# Autodesk Inventor assembly: Aux Cooling Assembly
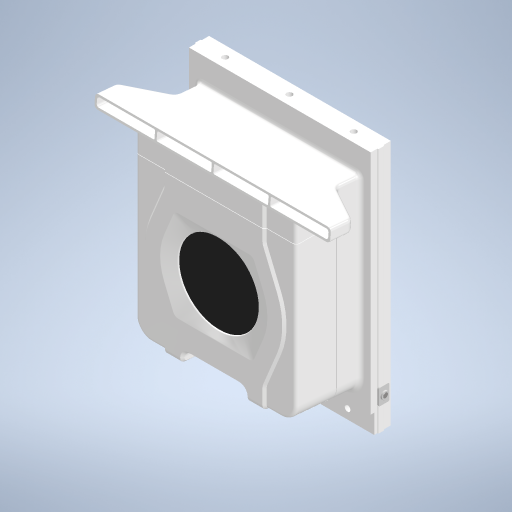
[picture p0: Inventor's stored thumbnail of the model, 512x512]
Saved by Autodesk Inventor 2024 (Build 280153000, 153)
## iProperties
Created: 2024-09-08
Part Number: Aux Cooling Assembly
Document SubType Name: Assembly
Designer: Ishaan
Author: Ishaan
## Documents named in this file (10)
- E:\Projects\Axiom--IDEX-3D-Printer\CAD\07 - Auxiliary Cooling\Aux Cooling Assembly.iam
- E:\Projects\Axiom--IDEX-3D-Printer\CAD\07 - Auxiliary Cooling\Aux Cooling Case.ipt
- E:\Projects\Axiom--IDEX-3D-Printer\CAD\00 - COTS Components\12032 Fan\SanAce_9BFB_120x32_BLW\SanAce_9BFB_120x32_BLW.ipt
- E:\Projects\Axiom--IDEX-3D-Printer\CAD\00 - COTS Components\HEPA Filter.ipt
- E:\Projects\Axiom--IDEX-3D-Printer\CAD\00 - COTS Components\Hardware\SHCSM5x20.ipt
- E:\Projects\Axiom--IDEX-3D-Printer\CAD\00 - COTS Components\Hardware\M5 LOCKNUT.ipt
- E:\Projects\Axiom--IDEX-3D-Printer\CAD\00 - COTS Components\Hardware\SHCSM5x16.ipt
- E:\Projects\Axiom--IDEX-3D-Printer\CAD\00 - COTS Components\Hardware\M5 T SLOT NUT.ipt
- E:\Projects\Axiom--IDEX-3D-Printer\CAD\00 - COTS Components\Hardware\SHCSM4x14.ipt
- E:\Projects\Axiom--IDEX-3D-Printer\CAD\00 - COTS Components\Hardware\M4 LOCKNUT.ipt
## Components (20 placed, 9 different names)
1. Aux Cooling Case:1 — Insert:1, Insert:2, Insert:3, Mate:1, Mate:2, Mate:3, Insert:4, Insert:5, Insert:6, Angle:1, Insert:7, Angle:2, Insert:8, Insert:9, Insert:10, Angle:3, Insert:11, Angle:4, Insert:12, Insert:13, Insert:14, Insert:18, Insert:19, Insert:20, Angle:5, Angle:6, Angle:7
2. SanAce_9BFB_120x32_BLW:1 — Insert:1, Insert:2, Insert:3, Insert:15, Insert:16, Insert:17
3. HEPA Filter:1 — Mate:1, Mate:2, Mate:3
4. SHCSM5x20:1 — Insert:4
5. SHCSM5x20:2 — Insert:5
6. M5 LOCKNUT:1 — Insert:7, Angle:2
7. M5 LOCKNUT:2 — Insert:6, Angle:1
8. SHCSM5x16:1 — Insert:8
9. SHCSM5x16:2 — Insert:9
10. M5 T SLOT NUT:1 — Insert:10, Angle:3
11. M5 T SLOT NUT:2 — Insert:11, Angle:4
12. SHCSM4x14:1 — Insert:12
13. SHCSM4x14:2 — Insert:13
14. SHCSM4x14:3 — Insert:14
15. M4 LOCKNUT:1 — Insert:15
16. M4 LOCKNUT:2 — Insert:17
17. M4 LOCKNUT:3 — Insert:16
18. M5 LOCKNUT:3 — Insert:20, Angle:5
19. M5 LOCKNUT:4 — Insert:19, Angle:6
20. M5 LOCKNUT:5 — Insert:18, Angle:7
## Relationships (30: Insert 20, Angle 7, Mate 3)
- Insert:1: Aux Cooling Case:1 ↔ SanAce_9BFB_120x32_BLW:1
- Insert:2: Aux Cooling Case:1 ↔ SanAce_9BFB_120x32_BLW:1
- Insert:3: Aux Cooling Case:1 ↔ SanAce_9BFB_120x32_BLW:1
- Mate:1 (0.5 mm): Aux Cooling Case:1 ↔ HEPA Filter:1
- Mate:2 (0.25 mm): Aux Cooling Case:1 ↔ HEPA Filter:1
- Mate:3 (0.5 mm): Aux Cooling Case:1 ↔ HEPA Filter:1
- Insert:4: Aux Cooling Case:1 ↔ SHCSM5x20:1
- Insert:5: Aux Cooling Case:1 ↔ SHCSM5x20:2
- Insert:6: Aux Cooling Case:1 ↔ M5 LOCKNUT:2
- Angle:1 (0 deg): Aux Cooling Case:1 ↔ M5 LOCKNUT:2
- Insert:7: Aux Cooling Case:1 ↔ M5 LOCKNUT:1
- Angle:2 (0 deg): Aux Cooling Case:1 ↔ M5 LOCKNUT:1
- Insert:8: Aux Cooling Case:1 ↔ SHCSM5x16:1
- Insert:9: Aux Cooling Case:1 ↔ SHCSM5x16:2
- Insert:10 (2 mm): Aux Cooling Case:1 ↔ M5 T SLOT NUT:1
- Angle:3 (0 deg): Aux Cooling Case:1 ↔ M5 T SLOT NUT:1
- Insert:11 (2 mm): Aux Cooling Case:1 ↔ M5 T SLOT NUT:2
- Angle:4 (0 deg): Aux Cooling Case:1 ↔ M5 T SLOT NUT:2
- Insert:12: Aux Cooling Case:1 ↔ SHCSM4x14:1
- Insert:13: Aux Cooling Case:1 ↔ SHCSM4x14:2
- Insert:14: Aux Cooling Case:1 ↔ SHCSM4x14:3
- Insert:15: SanAce_9BFB_120x32_BLW:1 ↔ M4 LOCKNUT:1
- Insert:16: SanAce_9BFB_120x32_BLW:1 ↔ M4 LOCKNUT:3
- Insert:17: SanAce_9BFB_120x32_BLW:1 ↔ M4 LOCKNUT:2
- Insert:18: Aux Cooling Case:1 ↔ M5 LOCKNUT:5
- Insert:19: Aux Cooling Case:1 ↔ M5 LOCKNUT:4
- Insert:20: Aux Cooling Case:1 ↔ M5 LOCKNUT:3
- Angle:5 (0 deg): Aux Cooling Case:1 ↔ M5 LOCKNUT:3
- Angle:6 (0 deg): Aux Cooling Case:1 ↔ M5 LOCKNUT:4
- Angle:7 (0 deg): Aux Cooling Case:1 ↔ M5 LOCKNUT:5
